# Autodesk Inventor assembly: stay1
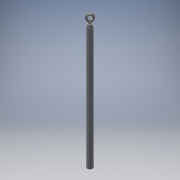
[picture p0: Inventor's stored thumbnail of the model, 180x180]
Saved by Autodesk Inventor 2018.2 (Build 222227000, 227)
## iProperties
Created: 2018-04-27
Part Number: stay1
Material: 一般
Document SubType Name: Assembly
Designer: ku_sk
Author: ku_sk
## Documents named in this file (3)
- Z:\各班フォルダ\2018\ボディ\エアロ\Aero\KS-15\Rr.wing\parts\stay\stay1.iam
- Z:\各班フォルダ\2018\ボディ\エアロ\Aero\KS-15\Rr.wing\parts\stay\pipe_16mm_360mm.ipt
- Z:\各班フォルダ\2018\ボディ\エアロ\Aero\KS-15\Rr.wing\parts\stay\end\stay end.iam
## Components (2 placed, 2 different names)
1. pipe_16mm_360mm:1 — メイト:1, メイト:2, メイト:3, メイト:4, メイト:5
2. stay end:1 [sub-assembly] — メイト:4, メイト:5
## Relationships (5: Mate 5)
- メイト:1 [Mate]: pipe_16mm_360mm:1
- メイト:2 [Mate]: pipe_16mm_360mm:1
- メイト:3 [Mate]: pipe_16mm_360mm:1
- メイト:4 [Mate]: pipe_16mm_360mm:1 ↔ stay end:1
- メイト:5 [Mate]: pipe_16mm_360mm:1 ↔ stay end:1
